# Autodesk Inventor assembly: Wrist2
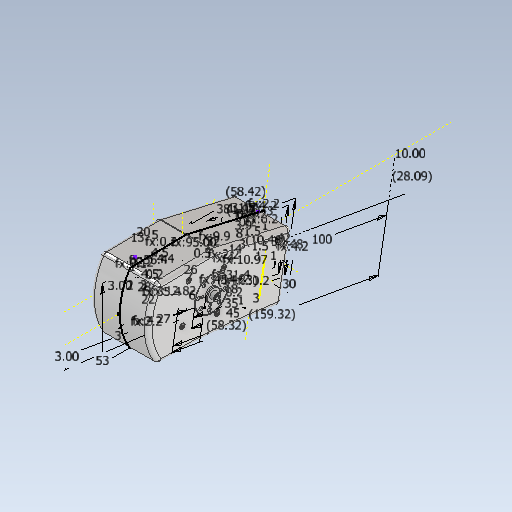
[picture p0: Inventor's stored thumbnail of the model, 512x512]
Saved by Autodesk Inventor 2021 (Build 250183000, 183)
## iProperties
Created: 2020-02-07
Part Number: Wrist2
Document SubType Name: Assembly
Designer: JochenAlt
Author: JochenAlt
## Documents named in this file (15)
- C:\Users\Jochen Alt\Documents\Daten\Projects\MiniBot\CAD\Wrist.iam
- C:\Users\Jochen Alt\Documents\Daten\Projects\MiniBot\CAD\extern\Herkulex\Herkulex DRS-040x.ipt
- C:\Users\Jochen Alt\Documents\Daten\Projects\MiniBot\CAD\extern\Herkulex\Herkulex DRS-020x.ipt
- C:\Users\Jochen Alt\Documents\Daten\Projects\MiniBot\CAD\extern\bearings\20x27x4\W 61704-2ZS.iam
- C:\Users\Jochen Alt\Documents\Daten\Projects\MiniBot\CAD\extern\bearings\25x32x4\W 61705-2RS1.iam
- C:\Users\Jochen Alt\Documents\Daten\Projects\MiniBot\CAD\Wrist.ipt
- C:\Users\Jochen Alt\Documents\Daten\Projects\MiniBot\CAD\WristFlange.ipt
- C:\Users\Jochen Alt\Documents\Daten\Projects\MiniBot\CAD\gripper\Base\Konstruktions-Assistent\Stirnzahnrad23.ipt
- D:\Projects\MiniBot\CAD\extern\DIN 912\DIN 912 - M2 x 0,4 x 6 x 5.ipt
- D:\Projects\MiniBot\CAD\extern\DIN 912\DIN 912 - M2 x 0.4 x 8 x 7.ipt
- D:\Projects\MiniBot\CAD\extern\DIN 912\DIN 912 - M2 x 0,4 x 20 x 19.ipt
- C:\Users\Jochen Alt\Documents\Daten\Projects\MiniBot\CAD\extern\accessories\Hex Spacer 10mm.ipt
- C:\Users\Jochen Alt\Documents\Inventor\Content Center Files\R2021\en-US\DIN 912\DIN 912 - M2 x 0.4 x 8 x 7.ipt
- C:\Users\Jochen Alt\Documents\Inventor\Content Center Files\R2021\en-US\DIN 934\DIN 934 - M2 x 0.4.ipt
- C:\Users\Jochen Alt\Documents\Daten\Projects\MiniBot\CAD\dimensions.xlsx
## Components (26 placed, 12 different names)
1. Herkulex DRS-0201:1 — Passend:28, Passend:30, Passend:42, Winkel:2, Passend:43, Mate:56, Mate:57
2. Herkulex DRS-040x:1 — Passend:36, Fluchtend:1, Winkel:1
3. W 61704-2ZS:2 [sub-assembly] — Mate:58, Mate:59
4. W 61705-2RS1:1 [sub-assembly] — Passend:32, Passend:37, Passend:46, Passend:47
5. Wrist:1 — Passend:32, Passend:36, Fluchtend:1, Winkel:1, Passend:37, Passend:42, Passend:43, Passend:48, Passend:49, Passend:50, Passend:51, Passend:52, Passend:53, Einfügen:1, Einfügen:2, Einfügen:3, Einfügen:4, Einfügen:5, Einfügen:6, Einfügen:7, Einfügen:8, Mate:58, Mate:59, Insert:9, Insert:10, Passend:60, Passend:61, Winkel:3
6. W 61705-2RS1:2 [sub-assembly]
7. WristFlange:1 — Passend:46, Passend:47, Insert:11, Insert:12, Insert:13, Mate:63
8. Stirnzahnrad2:1 — Mate:56, Mate:57
9. DIN 912 - replaced by DIN EN ISO 4762 M2 x 6:1 — Passend:48, Passend:49
10. DIN 912 - replaced by DIN EN ISO 4762 M2 x 6:2 — Passend:50, Passend:51
11. DIN 912 - replaced by DIN EN ISO 4762 M2 x 6:3 — Passend:52, Passend:53
12. DIN 912 - replaced by DIN EN ISO 4762 M2 x 8:1 — Einfügen:1
13. DIN 912 - replaced by DIN EN ISO 4762 M2 x 8:2 — Einfügen:2
14. DIN 912 - replaced by DIN EN ISO 4762 M2 x 8:3 — Einfügen:3
15. DIN 912 - replaced by DIN EN ISO 4762 M2 x 8:4 — Einfügen:4
16. DIN 912 - replaced by DIN EN ISO 4762 M2 x 8:5 — Einfügen:5
17. DIN 912 - replaced by DIN EN ISO 4762 M2 x 8:6 — Einfügen:6
18. DIN 912 - replaced by DIN EN ISO 4762 M2 x 8:7 — Einfügen:7
19. DIN 912 - replaced by DIN EN ISO 4762 M2 x 8:8 — Einfügen:8
20. DIN 912 - replaced by DIN EN ISO 4762 M2 x 20:1 — Insert:9
21. DIN 912 - replaced by DIN EN ISO 4762 M2 x 20:2 — Insert:10
22. Hex Spacer 10mm:1 — Passend:60, Passend:61, Winkel:3
23. DIN 912 - replaced by DIN EN ISO 4762 M2 x 8:9 — Insert:11, Mate:62
24. DIN 912 - replaced by DIN EN ISO 4762 M2 x 8:10 — Insert:12
25. DIN 912 - replaced by DIN EN ISO 4762 M2 x 8:11 — Insert:13
26. DIN 934 - replaced by DIN EN 24032/28673/28674 M2:1 — Mate:62, Mate:63
## Relationships (40: Mate 23, Insert 13, Angle 3, Flush 1)
- Passend:28 [Mate]: Herkulex DRS-0201:1
- Passend:30 [Mate]: Herkulex DRS-0201:1
- Passend:32 [Mate]: W 61705-2RS1:1 ↔ Wrist:1
- Passend:36 [Mate]: Herkulex DRS-040x:1 ↔ Wrist:1
- Fluchtend:1 [Flush]: Herkulex DRS-040x:1 ↔ Wrist:1
- Winkel:1 [Angle] (180 deg): Herkulex DRS-040x:1 ↔ Wrist:1
- Passend:37 [Mate] (0.1 mm): W 61705-2RS1:1 ↔ Wrist:1
- Passend:42 [Mate]: Herkulex DRS-0201:1 ↔ Wrist:1
- Winkel:2 [Angle] (180 deg): Herkulex DRS-0201:1
- Passend:43 [Mate] (0.2 mm): Herkulex DRS-0201:1 ↔ Wrist:1
- Passend:46 [Mate]: W 61705-2RS1:1 ↔ WristFlange:1
- Passend:47 [Mate]: W 61705-2RS1:1 ↔ WristFlange:1
- Passend:48 [Mate]: Wrist:1 ↔ DIN 912 - replaced by DIN EN ISO 4762 M2 x 6:1
- Passend:49 [Mate]: Wrist:1 ↔ DIN 912 - replaced by DIN EN ISO 4762 M2 x 6:1
- Passend:50 [Mate]: Wrist:1 ↔ DIN 912 - replaced by DIN EN ISO 4762 M2 x 6:2
- Passend:51 [Mate]: Wrist:1 ↔ DIN 912 - replaced by DIN EN ISO 4762 M2 x 6:2
- Passend:52 [Mate]: Wrist:1 ↔ DIN 912 - replaced by DIN EN ISO 4762 M2 x 6:3
- Passend:53 [Mate]: Wrist:1 ↔ DIN 912 - replaced by DIN EN ISO 4762 M2 x 6:3
- Einfügen:1 [Insert]: Wrist:1 ↔ DIN 912 - replaced by DIN EN ISO 4762 M2 x 8:1
- Einfügen:2 [Insert]: Wrist:1 ↔ DIN 912 - replaced by DIN EN ISO 4762 M2 x 8:2
- Einfügen:3 [Insert]: Wrist:1 ↔ DIN 912 - replaced by DIN EN ISO 4762 M2 x 8:3
- Einfügen:4 [Insert]: Wrist:1 ↔ DIN 912 - replaced by DIN EN ISO 4762 M2 x 8:4
- Einfügen:5 [Insert]: Wrist:1 ↔ DIN 912 - replaced by DIN EN ISO 4762 M2 x 8:5
- Einfügen:6 [Insert]: Wrist:1 ↔ DIN 912 - replaced by DIN EN ISO 4762 M2 x 8:6
- Einfügen:7 [Insert]: Wrist:1 ↔ DIN 912 - replaced by DIN EN ISO 4762 M2 x 8:7
- Einfügen:8 [Insert]: Wrist:1 ↔ DIN 912 - replaced by DIN EN ISO 4762 M2 x 8:8
- Mate:56: Herkulex DRS-0201:1 ↔ Stirnzahnrad2:1
- Mate:57: Herkulex DRS-0201:1 ↔ Stirnzahnrad2:1
- Mate:58: W 61704-2ZS:2 ↔ Wrist:1
- Mate:59: W 61704-2ZS:2 ↔ Wrist:1
- Insert:9: Wrist:1 ↔ DIN 912 - replaced by DIN EN ISO 4762 M2 x 20:1
- Insert:10: Wrist:1 ↔ DIN 912 - replaced by DIN EN ISO 4762 M2 x 20:2
- Passend:60 [Mate]: Wrist:1 ↔ Hex Spacer 10mm:1
- Passend:61 [Mate] (0.5 mm): Wrist:1 ↔ Hex Spacer 10mm:1
- Winkel:3 [Angle] (0 deg): Wrist:1 ↔ Hex Spacer 10mm:1
- Insert:11: WristFlange:1 ↔ DIN 912 - replaced by DIN EN ISO 4762 M2 x 8:9
- Insert:12: WristFlange:1 ↔ DIN 912 - replaced by DIN EN ISO 4762 M2 x 8:10
- Insert:13: WristFlange:1 ↔ DIN 912 - replaced by DIN EN ISO 4762 M2 x 8:11
- Mate:62: DIN 912 - replaced by DIN EN ISO 4762 M2 x 8:9 ↔ DIN 934 - replaced by DIN EN 24032/28673/28674 M2:1
- Mate:63: WristFlange:1 ↔ DIN 934 - replaced by DIN EN 24032/28673/28674 M2:1
## Named parameters: roundness_small = 3 mm, roundness_tiny = 0.5 mm, wall_thickness = 3 mm, medium_arm_width = 51 mm, big_arm_width = 56 mm, bevel_angle = 0.314159, medium_arm_radius = 35 mm, big_arm_radius = 48 mm, medium_arm_circle_centre = 11 mm, big_arm_circle_centre = 25 mm, thickness = 3 mm, tight_fit = 0.2 mm, press_fit = 0.1 mm, m2_screw_hole_diameter = 2.2 mm, m2_hex_width = 4.2 mm, m2_washer_diameter = 5.2 mm, m2_allen_screw_width = 4 mm, m2_allen_screw_height = 2 mm, m2_washer_height = 0.3 mm
note: some values were not read from the file. Shown as the stored number, unit unknown: "bevel_angle".
